# Autodesk Inventor assembly: SLIM_ASSEMBLED
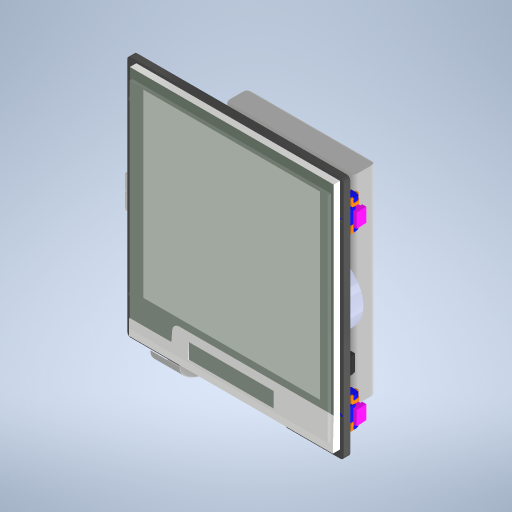
[picture p0: Inventor's stored thumbnail of the model, 512x512]
Saved by Autodesk Inventor 2023 (Build 270158000, 158)
## iProperties
Created: 2021-08-24
Part Number: SLIM_ASSEMBLED
Document SubType Name: Assembly
Designer: nigel
Author: nigel
## Documents named in this file (7)
- D:\NIGEL\Documents\GitHub\Watchy-CAD\CAD\Cases\SlimTouchscreenV1\SLIM_TC_ASSEMBLED_V1.iam
- D:\NIGEL\Documents\GitHub\Watchy-CAD\CAD\Base Model\WATCHY_CUT_TC.iam
- D:\NIGEL\Documents\GitHub\Watchy-CAD\CAD\Base Model\Battery_402535.ipt
- D:\NIGEL\Documents\GitHub\Watchy-CAD\CAD\Base Model\touch_pcb.ipt
- D:\NIGEL\Documents\GitHub\Watchy-CAD\CAD\Base Model\Battery_402030.ipt
- D:\NIGEL\Documents\GitHub\Watchy-CAD\CAD\Base Model\touch_panel_fpc.ipt
- D:\NIGEL\Documents\GitHub\Watchy-CAD\CAD\Cases\SlimV4\WatchyCaseParams.xlsx
## Components (5 placed, 5 different names)
1. WATCHY_CUT_TC:1 [sub-assembly] — Angle:1, Mate:11, Mate:12, Mate:13, Flush:9, Mate:16, Mate:17, Mate:18
2. Battery_402535:1 — Mate:11, Mate:18
3. touch_pcb:1 — Angle:1, Mate:14, Flush:8, Flush:10, Mate:15, Mate:16, Mate:17
4. Battery_402030:1 — Mate:12, Mate:13, Mate:15
5. touch_panel_fpc:1 — Mate:14, Flush:8, Flush:9, Flush:10
## Relationships (12: Mate 8, Flush 3, Angle 1)
- Angle:1 (180 deg): WATCHY_CUT_TC:1 ↔ touch_pcb:1
- Mate:11: WATCHY_CUT_TC:1 ↔ Battery_402535:1
- Mate:12 (0.5 mm): WATCHY_CUT_TC:1 ↔ Battery_402030:1
- Mate:13: WATCHY_CUT_TC:1 ↔ Battery_402030:1
- Mate:14 (0.5 mm): touch_pcb:1 ↔ touch_panel_fpc:1
- Flush:8: touch_pcb:1 ↔ touch_panel_fpc:1
- Flush:9: WATCHY_CUT_TC:1 ↔ touch_panel_fpc:1
- Flush:10 (3.8 mm): touch_pcb:1 ↔ touch_panel_fpc:1
- Mate:15 (0.5 mm): touch_pcb:1 ↔ Battery_402030:1
- Mate:16: WATCHY_CUT_TC:1 ↔ touch_pcb:1
- Mate:17: WATCHY_CUT_TC:1 ↔ touch_pcb:1
- Mate:18 (0.5 mm): WATCHY_CUT_TC:1 ↔ Battery_402535:1
## Named parameters: pcb_thickness = 0.94 mm, case_thickness = 1 mm, electronics_thickness = 6.4 mm, usb_height = 4 mm, strap_pin_depth = 2.3 mm, top_thickness = 0.2 mm, display_thickness = 1.2 mm
